# Autodesk Inventor assembly: box assembly
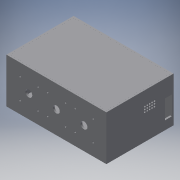
[picture p0: Inventor's stored thumbnail of the model, 180x180]
Saved by Autodesk Inventor 2018 (Build 220112000, 112)
## iProperties
Created: 2018-05-15
Part Number: box assembly
Document SubType Name: Assembly
Designer: Administrator
Author: Administrator
## Documents named in this file (6)
- H:\Projects\box assembly.iam
- H:\Projects\top.ipt
- H:\Projects\hole side.ipt
- H:\Projects\other hole side.ipt
- H:\Projects\basic side.ipt
- H:\Projects\bottom.ipt
## Components (6 placed, 5 different names)
1. top:1 — Mate:1, Flush:1, Flush:2, Mate:2, Flush:3, Flush:4, Flush:5, Mate:4
2. hole side:1 — Mate:1, Flush:1, Flush:2, Mate:3, Flush:6, Flush:7, Flush:8
3. other hole side:1 — Mate:2, Flush:3, Flush:4, Mate:5
4. basic side:1 — Flush:5, Mate:3, Flush:6, Mate:6
5. basic side:2 — Flush:7, Mate:4, Mate:5, Flush:9
6. bottom:1 — Flush:8, Mate:6, Flush:9
## Relationships (15: Flush 9, Mate 6)
- Mate:1: top:1 ↔ hole side:1
- Flush:1: top:1 ↔ hole side:1
- Flush:2: top:1 ↔ hole side:1
- Mate:2: top:1 ↔ other hole side:1
- Flush:3: top:1 ↔ other hole side:1
- Flush:4: top:1 ↔ other hole side:1
- Flush:5: top:1 ↔ basic side:1
- Mate:3: hole side:1 ↔ basic side:1
- Flush:6: hole side:1 ↔ basic side:1
- Flush:7: hole side:1 ↔ basic side:2
- Mate:4: top:1 ↔ basic side:2
- Mate:5: other hole side:1 ↔ basic side:2
- Flush:8: hole side:1 ↔ bottom:1
- Mate:6: basic side:1 ↔ bottom:1
- Flush:9: basic side:2 ↔ bottom:1
